# Autodesk Inventor assembly: Conjunto Ambu
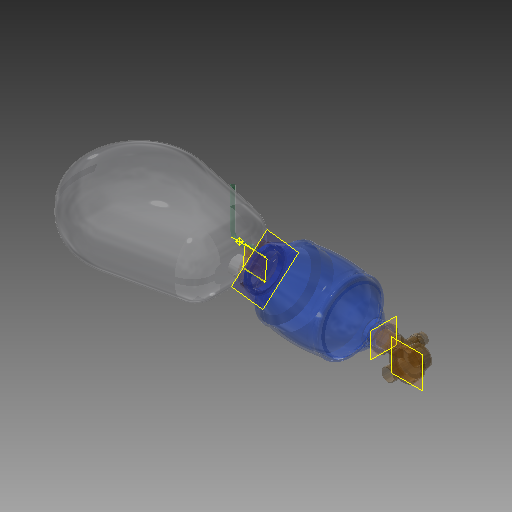
[picture p0: Inventor's stored thumbnail of the model, 512x512]
Saved by Autodesk Inventor 2019 (Build 230136000, 136)
## iProperties
Created: 2020-04-02
Part Number: Conjunto Ambu
Material: Genérico
Document SubType Name: Assembly
Designer: Paulo Rodrigues
Author: Paulo Rodrigues
## Documents named in this file (10)
- E:\COVID19\Respirador V3\Conjunto Ambu.iam
- E:\COVID19\Respirador V3\Corpo do Ambu.ipt
- E:\COVID19\Respirador V3\Tampa de Entrada.ipt
- E:\COVID19\Respirador V3\Bolsa de Carregamento.ipt
- E:\COVID19\Respirador V3\Adaptador de Saida.ipt
- E:\COVID19\Respirador V3\Corpo Valvula de Saida.ipt
- E:\COVID19\Respirador V3\Bocal de Saída.ipt
- E:\COVID19\Respirador V3\Corpo Valvula Reguladora de Pressão.ipt
- E:\COVID19\Respirador V3\Pino de Liberação Valvula Alivio de Pressão.ipt
- E:\COVID19\Respirador V3\Tubo de Entrada do Ar.ipt
## Components (9 placed, 9 different names)
1. Corpo do Ambu:1 — Alinhamento:1, Alinhamento:2, Alinhamento:3, Alinhamento:4, Ângulo:2, Inserir:2, Ângulo:3
2. Tampa de Entrada:1 — Alinhamento:1, Alinhamento:2, Inserir:1, Coincidência:1, Coincidência:2, Inserir:2, Inserir:4
3. Bolsa de Carregamento:2 — Inserir:1, Ângulo:1
4. Adaptador de Saida:1 — Alinhamento:3, Alinhamento:4, Inserir:3
5. Corpo Valvula de Saida:1 — Inserir:3, Ângulo:3, Alinhamento:5, Alinhamento:6, Alinhamento:7
6. Bocal de Saída:1 — Alinhamento:5, Alinhamento:6
7. Corpo Valvula Reguladora de Pressão:1 — Alinhamento:7, Alinhamento:8
8. Pino de Liberação Valvula Alivio de Pressão:1 — Alinhamento:8
9. Tubo de Entrada do Ar:2 — Inserir:4
## Relationships (19: Flush 8, Insert 4, Mate 4, Angle 3)
- Alinhamento:1 [Flush]: Corpo do Ambu:1 ↔ Tampa de Entrada:1
- Alinhamento:2 [Flush]: Corpo do Ambu:1 ↔ Tampa de Entrada:1
- Inserir:1 (-15 mm): Tampa de Entrada:1 ↔ Bolsa de Carregamento:2
- Coincidência:1 [Mate]: Tampa de Entrada:1
- Coincidência:2 [Mate]: Tampa de Entrada:1
- Coincidência:3 [Mate]
- Coincidência:4 [Mate]
- Ângulo:1 [Angle] (90 deg): Bolsa de Carregamento:2
- Alinhamento:3 [Flush]: Corpo do Ambu:1 ↔ Adaptador de Saida:1
- Alinhamento:4 [Flush]: Corpo do Ambu:1 ↔ Adaptador de Saida:1
- Ângulo:2 [Angle] (0 deg): Corpo do Ambu:1
- Inserir:2: Corpo do Ambu:1 ↔ Tampa de Entrada:1
- Inserir:3 (-10 mm): Adaptador de Saida:1 ↔ Corpo Valvula de Saida:1
- Ângulo:3 [Angle] (0 deg): Corpo do Ambu:1 ↔ Corpo Valvula de Saida:1
- Alinhamento:5 [Flush]: Corpo Valvula de Saida:1 ↔ Bocal de Saída:1
- Alinhamento:6 [Flush]: Corpo Valvula de Saida:1 ↔ Bocal de Saída:1
- Alinhamento:7 [Flush]: Corpo Valvula de Saida:1 ↔ Corpo Valvula Reguladora de Pressão:1
- Alinhamento:8 [Flush]: Corpo Valvula Reguladora de Pressão:1 ↔ Pino de Liberação Valvula Alivio de Pressão:1
- Inserir:4: Tampa de Entrada:1 ↔ Tubo de Entrada do Ar:2
